# Autodesk Inventor assembly: plateau_mobile_servos
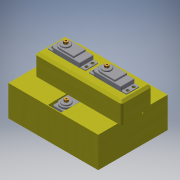
[picture p0: Inventor's stored thumbnail of the model, 180x180]
Saved by Autodesk Inventor 2018 (Build 220112000, 112)
## iProperties
Created: 2017-10-12
Part Number: plateau_mobile_servos
Document SubType Name: Assembly
Designer: liamg
Author: liamg
## Documents named in this file (4)
- C:\Users\liamg\Desktop\Rotor\socle coulissant\plateau_mobile_servos.iam
- C:\Users\liamg\Desktop\Rotor\socle coulissant\Socle servo.ipt
- C:\Users\liamg\Desktop\Rotor\socle coulissant\plateau_coulisseant.ipt
- C:\Users\liamg\Desktop\Rotor\Servo moteur\servo.iam
## Components (5 placed, 3 different names)
1. Socle servo:1 — Flush:1, Slider:1, Insert:1, Insert:2, Insert:3, Insert:4
2. plateau_coulisseant:1 — Flush:1, Slider:1, Insert:5, Insert:6
3. servo:1 [sub-assembly] — Insert:3, Insert:4
4. servo:2 [sub-assembly] — Insert:1, Insert:2
5. servo:3 [sub-assembly] — Insert:5, Insert:6
## Relationships (8: Insert 6, Flush 1, TranslationJoint 1)
- Flush:1: Socle servo:1 ↔ plateau_coulisseant:1
- Slider:1 [TranslationJoint]: Socle servo:1 ↔ plateau_coulisseant:1
- Insert:1: Socle servo:1 ↔ servo:2
- Insert:2: Socle servo:1 ↔ servo:2
- Insert:3: Socle servo:1 ↔ servo:1
- Insert:4: Socle servo:1 ↔ servo:1
- Insert:5: plateau_coulisseant:1 ↔ servo:3
- Insert:6: plateau_coulisseant:1 ↔ servo:3
